# Autodesk Inventor assembly: A
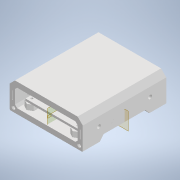
[picture p0: Inventor's stored thumbnail of the model, 180x180]
Saved by Autodesk Inventor 2022.2 (Build 262287000, 287)
## iProperties
Created: 2021-12-01
Part Number: A
Document SubType Name: Assembly
Designer: kfcs7
Author: kfcs7
## Documents named in this file (4)
- C:\Users\kfcs7\Desktop\Differential-Signal-Generator\models\A.iam
- C:\Users\kfcs7\Desktop\Differential-Signal-Generator\models\A-00.ipt
- C:\Users\kfcs7\Desktop\Differential-Signal-Generator\models\A-01.ipt
- C:\Users\kfcs7\Desktop\Differential-Signal-Generator\models\A-02.ipt
## Components (3 placed, 3 different names)
1. A-00:1 — Mate:1, Mate:2, Mate:3
2. A-01:1 — Mate:1, Mate:2, Mate:3
3. A-02:1
## Relationships (3: Mate 3)
- Mate:1: A-00:1 ↔ A-01:1
- Mate:2: A-00:1 ↔ A-01:1
- Mate:3: A-00:1 ↔ A-01:1
